# Autodesk Inventor assembly: 000 Ensamblaje hw_LM - BASIC
(part 4 of 4)
- Mate:289: Cooling Kit for NVIDIA Jetson Xavier NX - screws-harness:1 ↔ P3767-pcba-envelop_20230310-modificada:1
## Named parameters: d178_d163 = 0 mm, d193_d188 = 0 mm, d196_d184 = 0 mm, d203_d178_d163 = 0 mm, d205_d180 = 0 mm, d231_d187 = 0 mm, d239_d202_d177_d162 = 0 mm, d304_d302 = 0 mm, d308_d306 = 0 mm, d309_d307 = 0 mm, d310_d304_d302 = 0 mm, d313_d307 = 0 mm, d316_d237_d198_d178_d163 = 0 mm, d317_d238_d200_d180 = 0 mm, d323_d316_d237_d198_d178_d163 = 0 mm, d324_d317_d238_d200_d180 = 0 mm, d325_d318_d240_d203_d178_d163 = 0 mm, d326_d319_d242_d205_d180 = 0 mm, d327_d320_d243_d206 = 0 mm, d328_d321 = 0 mm, d331_d323_d316_d237_d198_d178_d163 = 0 mm, d332_d324_d317_d238_d200_d180 = 0 mm, d337_d322 = 0 mm, d421_d415 = 0 mm, d457_d340 = 0 mm, d464_d457_d340 = 0 mm, d465_d458 = 0 mm, d467_d460 = 0 mm, d471_d456_d340 = 0 mm, d472_d457_d340 = 0 mm, d474_d459 = 0 mm, d477_d463_d456_d340 = 0 mm, d488_d471_d456_d340 = 0 mm, d489_d472_d457_d340 = 0 mm, d490_d473_d458 = 0 mm, d491_d474_d459 = 0 mm, d492_d475_d460 = 0 mm, d493_d476_d461 = 0 mm, d494_d477_d463_d456_d340 = 0 mm, d495_d478_d464_d457_d340 = 0 mm, d496_d479_d465_d458 = 0 mm, d497_d480_d466_d459 = 0 mm, d498_d481_d467_d460 = 0 mm, d499_d482_d468_d461 = 0 mm, d500_d483_d469 = 0 mm, d501_d484_d470 = 0 mm, d502_d486 = 0 mm, d506_d471_d456_d340 = 0 mm, d507_d489_d472_d457_d340 = 0 mm, d508_d490_d473_d458 = 0 mm, d509_d492_d475_d460 = 0 mm, d510_d495_d478_d464_d457_d340 = 0 mm, d511_d496_d479_d465_d458 = 0 mm, d512_d498_d481_d467_d460 = 0 mm, d513_d502_d486 = 0 mm, d514_d503 = 0 mm, d515_d504 = 0 mm, d516_d471_d456_d340 = 0 mm, d520_d495_d478_d464_d457_d340 = 0 mm, d521_d496_d479_d465_d458 = 0 mm, d522_d498_d481_d467_d460 = 0 mm, d524_d503 = 0 mm, d525_d504 = 0 mm, d576_d508_d490_d473_d458 = 0 mm, d591_d581_d575_d507_d489_d472_d457_d340 = 0 mm, d592_d582_d576_d508_d490_d473_d458 = 0 mm, d593_d583_d577_d509_d492_d475_d460 = 0 mm, d594_d584_d578 = 0 mm, d595_d585_d579 = 0 mm, d596_d586_d580 = 0 mm, d597_d589 = 0 mm, d598_d590 = 0 mm, d599_d581_d575_d507_d489_d472_d457_d340 = 0 mm, d600_d582_d576_d508_d490_d473_d458 = 0 mm, d601_d583_d577_d509_d492_d475_d460 = 0 mm, d602_d584_d578 = 0 mm, d603_d585_d579 = 0 mm, d604_d586_d580 = 0 mm, d605_d589 = 0 mm, d606_d590 = 0 mm, d608_d592_d582_d576_d508_d490_d473_d458 = 0 mm, d609_d593_d583_d577_d509_d492_d475_d460 = 0 mm, d611_d595_d585_d579 = 0 mm, d612_d596_d586_d580 = 0 mm, d613_d597_d589 = 0 mm, d614_d598_d590 = 0 mm, d632_d599_d581_d575_d507_d489_d472_d457_d340 = 0 mm, d635_d602_d584_d578 = 0 mm, d638_d605_d589 = 0 mm, d639_d606_d590 = 0 mm, d640_d623 = 0 deg, d644_d627 = 0 deg, d645_d628 = 0 deg, d650_d581_d575_d507_d489_d472_d457_d340 = 0 mm, d651_d582_d576_d508_d490_d473_d458 = 0 mm, d652_d446_d178_d163 = 0 mm, d653_d447_d180 = 0 mm, d654_d449 = 0 mm, d655_d452 = 0 mm, d682_d678 = 0 mm, d683_d679 = 0 mm, d684_d680 = 0 mm, d737_d728 = 0 mm, d738_d730 = 0 mm, d739_d731 = 0 mm, d740_d732 = 0 mm, d746_d737_d728 = 0 mm, d747_d738_d730 = 0 mm, d748_d739_d731 = 0 mm, d749_d740_d732 = 0 mm, d750_d737_d728 = 0 mm, d751_d738_d730 = 0 mm, d752_d739_d731 = 0 mm, d753_d740_d732 = 0 mm, d762_d753_d740_d732 = 0 mm, d766_d753_d740_d732 = 0 mm, d775_d763_d750_d737_d728 = 0 mm, d776_d764_d751_d738_d730 = 0 mm, d777_d765_d752_d739_d731 = 0 mm, d778_d766_d753_d740_d732 = 0 mm, d783_d775_d763_d750_d737_d728 = 0 mm, d784_d777_d765_d752_d739_d731 = 0 mm, d785_d778_d766_d753_d740_d732 = 0 mm, d786_d775_d763_d750_d737_d728 = 0 mm, d787_d777_d765_d752_d739_d731 = 0 mm, d788_d778_d766_d753_d740_d732 = 0 mm, d798_d775_d763_d750_d737_d728 = 0 mm, d799_d786_d775_d763_d750_d737_d728 = 0 mm, d800_d787_d777_d765_d752_d739_d731 = 0 mm, d801_d788_d778_d766_d753_d740_d732 = 0 mm, d802_d790 = 0 deg, d803_d793 = 0 deg, d804_d794 = 0 deg, d810_d786_d775_d763_d750_d737_d728 = 0 mm, d811_d787_d777_d765_d752_d739_d731 = 0 mm, d812_d788_d778_d766_d753_d740_d732 = 0 mm, d814_d793 = 0 deg, d815_d794 = 0 deg, d816_d798_d775_d763_d750_d737_d728 = 0 mm, d817_d799_d786_d775_d763_d750_d737_d728 = 0 mm, d818_d800_d787_d777_d765_d752_d739_d731 = 0 mm, d819_d801_d788_d778_d766_d753_d740_d732 = 0 mm, d820_d802_d790 = 0 deg, d821_d803_d793 = 0 deg, d822_d804_d794 = 0 deg, d823_d805 = 0 mm, d824_d806 = 0 mm, d825_d807 = 0 mm, d836_d829 = 0 mm, d839_d810_d786_d775_d763_d750_d737_d728 = 0 mm, d840_d811_d787_d777_d765_d752_d739_d731 = 0 mm, d841_d812_d788_d778_d766_d753_d740_d732 = 0 mm, d842_d814_d793 = 0 deg, d843_d815_d794 = 0 deg, d844_d817_d799_d786_d775_d763_d750_d737_d728 = 0 mm, d845_d818_d800_d787_d777_d765_d752_d739_d731 = 0 mm, d846_d819_d801_d788_d778_d766_d753_d740_d732 = 0 mm, d847_d821_d803_d793 = 0 deg, d848_d822_d804_d794 = 0 deg, d856_d836_d829 = 0 mm, d857_d837_d775_d763_d750_d737_d728 = 0 mm, d858_d838_d790 = 0 deg, d859_d839_d810_d786_d775_d763_d750_d737_d728 = 0 mm, d860_d840_d811_d787_d777_d765_d752_d739_d731 = 0 mm, d861_d841_d812_d788_d778_d766_d753_d740_d732 = 0 mm, d862_d842_d814_d793 = 0 deg, d863_d843_d815_d794 = 0 deg, d867_d847_d821_d803_d793 = 0 deg, d868_d848_d822_d804_d794 = 0 deg, d870_d851 = 0 mm, d871_d852 = 0 mm, d872_d853 = 0 mm, d886_d883 = 0 mm, d888_d885 = 0 mm, d889_d878 = 0 deg, d890_d880_d878 = 0 deg, d892_d882_d847_d821_d803_d793 = 0 deg, d899_d878 = 0 deg, d901_d847_d821_d803_d793 = 0 deg, d906_d878 = 0 deg, d908_d847_d821_d803_d793 = 0 deg, d1127_d395 = 0 mm, d1128_d396 = 0 mm, d1129_d397 = 0 mm, d1215_d178_d163 = 0 mm, d1216_d180 = 0 mm, d1234_d1229 = 0 mm, d1235_d1230 = 0 mm, d1236_d1231 = 0 mm, d1237_d1232 = 0 mm, d1238_d1233 = 0 mm, d1243_d1241 = 0 mm, d1244_d1242 = 0 mm, d1245_d1229 = 0 mm, d1246_d1230 = 0 mm, d1247_d1231 = 0 mm, d1248_d1232 = 0 mm, d1249_d1233 = 0 mm, d1250_d1234_d1229 = 0 mm, d1251_d1235_d1230 = 0 mm, d1252_d1236_d1231 = 0 mm, d1253_d1237_d1232 = 0 mm, d1254_d1238_d1233 = 0 mm, d1255_d1239 = 0 mm, d1260_d1241 = 0 mm, d1261_d1242 = 0 mm, d1262_d1229 = 0 mm, d1263_d1230 = 0 mm, d1264_d1231 = 0 mm, d1265_d1232 = 0 mm, d1266_d1233 = 0 mm, d1267_d1234_d1229 = 0 mm, d1268_d1235_d1230 = 0 mm, d1269_d1236_d1231 = 0 mm, d1270_d1237_d1232 = 0 mm, d1271_d1238_d1233 = 0 mm, d1272_d1239 = 0 mm, d1273_d1260_d1241 = 0 mm, d1274_d1261_d1242 = 0 mm, d1275_d1262_d1229 = 0 mm, d1276_d1263_d1230 = 0 mm, d1277_d1264_d1231 = 0 mm, d1278_d1265_d1232 = 0 mm, d1279_d1266_d1233 = 0 mm, d1280_d1267_d1234_d1229 = 0 mm, d1281_d1268_d1235_d1230 = 0 mm, d1282_d1269_d1236_d1231 = 0 mm, d1283_d1272_d1239 = 0 mm, d1288_d1260_d1241 = 0 mm, d1289_d1261_d1242 = 0 mm, d1290_d1262_d1229 = 0 mm, d1291_d1263_d1230 = 0 mm, d1292_d1264_d1231 = 0 mm, d1293_d1265_d1232 = 0 mm, d1294_d1266_d1233 = 0 mm, d1295_d1267_d1234_d1229 = 0 mm, d1296_d1268_d1235_d1230 = 0 mm, d1297_d1269_d1236_d1231 = 0 mm, d1298_d1272_d1239 = 0 mm, d1299_d1274_d1261_d1242 = 0 mm, d1300_d1275_d1262_d1229 = 0 mm, d1301_d1276_d1263_d1230 = 0 mm, d1302_d1277_d1264_d1231 = 0 mm, d1303_d1278_d1265_d1232 = 0 mm, d1304_d1279_d1266_d1233 = 0 mm, d1305_d1280_d1267_d1234_d1229 = 0 mm, d1306_d1283_d1272_d1239 = 0 mm, d1307_d1288_d1260_d1241 = 0 mm, d1308_d1289_d1261_d1242 = 0 mm, d1309_d1290_d1262_d1229 = 0 mm, d1310_d1291_d1263_d1230 = 0 mm, d1311_d1292_d1264_d1231 = 0 mm, d1312_d1293_d1265_d1232 = 0 mm, d1313_d1294_d1266_d1233 = 0 mm, d1314_d1295_d1267_d1234_d1229 = 0 mm, d1315_d1296_d1268_d1235_d1230 = 0 mm, d1316_d1297_d1269_d1236_d1231 = 0 mm, d1317_d1298_d1272_d1239 = 0 mm, d1324_d1321 = 0 mm, d1325_d1323 = 0 mm, d1326_d1300_d1275_d1262_d1229 = 0 mm, d1327_d1301_d1276_d1263_d1230 = 0 mm, d1328_d1302_d1277_d1264_d1231 = 0 mm, d1329_d1303_d1278_d1265_d1232 = 0 mm, d1330_d1304_d1279_d1266_d1233 = 0 mm, d1331_d1307_d1288_d1260_d1241 = 0 mm, d1332_d1308_d1289_d1261_d1242 = 0 mm, d1333_d1309_d1290_d1262_d1229 = 0 mm, d1334_d1310_d1291_d1263_d1230 = 0 mm, d1335_d1311_d1292_d1264_d1231 = 0 mm, d1336_d1312_d1293_d1265_d1232 = 0 mm, d1337_d1313_d1294_d1266_d1233 = 0 mm, d1338_d1314_d1295_d1267_d1234_d1229 = 0 mm, d1339_d1315_d1296_d1268_d1235_d1230 = 0 mm, d1340_d1316_d1297_d1269_d1236_d1231 = 0 mm, d1341_d1317_d1298_d1272_d1239 = 0 mm, d1350_d1324_d1321 = 0 mm, d1351_d1325_d1323 = 0 mm, d1352_d1326_d1300_d1275_d1262_d1229 = 0 mm, d1353_d1327_d1301_d1276_d1263_d1230 = 0 mm, d1354_d1328_d1302_d1277_d1264_d1231 = 0 mm, d1355_d1329_d1303_d1278_d1265_d1232 = 0 mm, d1356_d1330_d1304_d1279_d1266_d1233 = 0 mm, d1357_d1331_d1307_d1288_d1260_d1241 = 0 mm, d1358_d1332_d1308_d1289_d1261_d1242 = 0 mm, d1359_d1333_d1309_d1290_d1262_d1229 = 0 mm, d1360_d1334_d1310_d1291_d1263_d1230 = 0 mm, d1361_d1335_d1311_d1292_d1264_d1231 = 0 mm, d1362_d1336_d1312_d1293_d1265_d1232 = 0 mm, d1363_d1337_d1313_d1294_d1266_d1233 = 0 mm, d1364_d1338_d1314_d1295_d1267_d1234_d1229 = 0 mm, d1365_d1339_d1315_d1296_d1268_d1235_d1230 = 0 mm, d1366_d1340_d1316_d1297_d1269_d1236_d1231 = 0 mm, d1367_d1341_d1317_d1298_d1272_d1239 = 0 mm, d1370_d1363_d1337_d1313_d1294_d1266_d1233 = 0 mm, d1377_d1370_d1363_d1337_d1313_d1294_d1266_d1233 = 0 mm, d1378_d1372 = 0 deg, d1379_d1373 = 0 deg, d1380_d1374 = 0 mm, d1381_d1375 = 0 mm, d1382_d1370_d1363_d1337_d1313_d1294_d1266_d1233 = 0 mm, d1383_d1372 = 0 deg, d1384_d1373 = 0 deg, d1385_d1374 = 0 mm, d1386_d1375 = 0 mm, d1391_d1370_d1363_d1337_d1313_d1294_d1266_d1233 = 0 mm, d1392_d1372 = 0 deg, d1393_d1373 = 0 deg, d1394_d1374 = 0 mm, d1395_d1375 = 0 mm, d1397_d1378_d1372 = 0 deg, d1398_d1379_d1373 = 0 deg, d1399_d1380_d1374 = 0 mm, d1400_d1381_d1375 = 0 mm, d1402_d1383_d1372 = 0 deg, d1403_d1384_d1373 = 0 deg, d1404_d1385_d1374 = 0 mm, d1405_d1386_d1375 = 0 mm, d1406_d1387 = 0 mm, d1407_d1388 = 0 mm, d1408_d1389 = 0 mm, d1409_d1390 = 0 mm, d1410_d1370_d1363_d1337_d1313_d1294_d1266_d1233 = 0 mm, d1411_d1372 = 0 deg, d1412_d1373 = 0 deg, d1413_d1374 = 0 mm, d1414_d1375 = 0 mm, d1416_d1378_d1372 = 0 deg, d1417_d1379_d1373 = 0 deg, d1418_d1380_d1374 = 0 mm, d1419_d1381_d1375 = 0 mm, d1421_d1383_d1372 = 0 deg, d1422_d1384_d1373 = 0 deg, d1423_d1385_d1374 = 0 mm, d1424_d1386_d1375 = 0 mm, d1425_d1387 = 0 mm, d1426_d1388 = 0 mm, d1427_d1389 = 0 mm, d1428_d1390 = 0 mm, d1433_d1411_d1372 = 0 deg, d1434_d1412_d1373 = 0 deg, d1435_d1413_d1374 = 0 mm, d1436_d1414_d1375 = 0 mm, d1438_d1416_d1378_d1372 = 0 deg, d1439_d1417_d1379_d1373 = 0 deg, d1440_d1418_d1380_d1374 = 0 mm, d1441_d1419_d1381_d1375 = 0 mm, d1443_d1421_d1383_d1372 = 0 deg, d1444_d1422_d1384_d1373 = 0 deg, d1445_d1423_d1385_d1374 = 0 mm, d1446_d1424_d1386_d1375 = 0 mm, d1447_d1425_d1387 = 0 mm, d1448_d1426_d1388 = 0 mm, d1449_d1427_d1389 = 0 mm, d1450_d1428_d1390 = 0 mm, d1452_d1411_d1372 = 0 deg, d1453_d1412_d1373 = 0 deg, d1454_d1413_d1374 = 0 mm, d1455_d1414_d1375 = 0 mm, d1457_d1416_d1378_d1372 = 0 deg, d1458_d1417_d1379_d1373 = 0 deg, d1459_d1418_d1380_d1374 = 0 mm, d1460_d1419_d1381_d1375 = 0 mm, d1462_d1421_d1383_d1372 = 0 deg, d1463_d1422_d1384_d1373 = 0 deg, d1464_d1423_d1385_d1374 = 0 mm, d1465_d1424_d1386_d1375 = 0 mm, d1466_d1425_d1387 = 0 mm, d1467_d1426_d1388 = 0 mm, d1468_d1427_d1389 = 0 mm, d1469_d1428_d1390 = 0 mm, d1474_d1433_d1411_d1372 = 0 deg, d1475_d1434_d1412_d1373 = 0 deg, d1476_d1435_d1413_d1374 = 0 mm, d1477_d1436_d1414_d1375 = 0 mm, d1479_d1438_d1416_d1378_d1372 = 0 deg, d1480_d1439_d1417_d1379_d1373 = 0 deg, d1481_d1440_d1418_d1380_d1374 = 0 mm, d1482_d1441_d1419_d1381_d1375 = 0 mm, d1484_d1443_d1421_d1383_d1372 = 0 deg, d1485_d1444_d1422_d1384_d1373 = 0 deg, d1486_d1445_d1423_d1385_d1374 = 0 mm, d1487_d1446_d1424_d1386_d1375 = 0 mm, d1488_d1447_d1425_d1387 = 0 mm, d1489_d1448_d1426_d1388 = 0 mm, d1490_d1449_d1427_d1389 = 0 mm, d1491_d1450_d1428_d1390 = 0 mm, d1493_d1433_d1411_d1372 = 0 deg, d1494_d1434_d1412_d1373 = 0 deg, d1495_d1435_d1413_d1374 = 0 mm, d1496_d1436_d1414_d1375 = 0 mm, d1498_d1438_d1416_d1378_d1372 = 0 deg, d1499_d1439_d1417_d1379_d1373 = 0 deg, d1500_d1440_d1418_d1380_d1374 = 0 mm, d1501_d1441_d1419_d1381_d1375 = 0 mm, d1503_d1443_d1421_d1383_d1372 = 0 deg, d1504_d1444_d1422_d1384_d1373 = 0 deg, d1505_d1445_d1423_d1385_d1374 = 0 mm, d1506_d1446_d1424_d1386_d1375 = 0 mm, d1507_d1447_d1425_d1387 = 0 mm, d1508_d1448_d1426_d1388 = 0 mm, d1509_d1449_d1427_d1389 = 0 mm, d1510_d1450_d1428_d1390 = 0 mm, d1516_d1493_d1433_d1411_d1372 = 0 deg, d1517_d1494_d1434_d1412_d1373 = 0 deg, d1518_d1495_d1435_d1413_d1374 = 0 mm, d1519_d1496_d1436_d1414_d1375 = 0 mm, d1521_d1498_d1438_d1416_d1378_d1372 = 0 deg, d1522_d1499_d1439_d1417_d1379_d1373 = 0 deg, d1523_d1500_d1440_d1418_d1380_d1374 = 0 mm, d1524_d1501_d1441_d1419_d1381_d1375 = 0 mm, d1526_d1503_d1443_d1421_d1383_d1372 = 0 deg, d1527_d1504_d1444_d1422_d1384_d1373 = 0 deg, d1528_d1505_d1445_d1423_d1385_d1374 = 0 mm, d1529_d1506_d1446_d1424_d1386_d1375 = 0 mm, d1530_d1507_d1447_d1425_d1387 = 0 mm, d1531_d1508_d1448_d1426_d1388 = 0 mm, d1532_d1509_d1449_d1427_d1389 = 0 mm, d1533_d1510_d1450_d1428_d1390 = 0 mm, d1535_d1493_d1433_d1411_d1372 = 0 deg, d1536_d1494_d1434_d1412_d1373 = 0 deg, d1537_d1495_d1435_d1413_d1374 = 0 mm, d1538_d1496_d1436_d1414_d1375 = 0 mm, d1540_d1498_d1438_d1416_d1378_d1372 = 0 deg, d1541_d1499_d1439_d1417_d1379_d1373 = 0 deg, d1542_d1500_d1440_d1418_d1380_d1374 = 0 mm, d1543_d1501_d1441_d1419_d1381_d1375 = 0 mm, d1545_d1503_d1443_d1421_d1383_d1372 = 0 deg, d1546_d1504_d1444_d1422_d1384_d1373 = 0 deg, d1547_d1505_d1445_d1423_d1385_d1374 = 0 mm, d1548_d1506_d1446_d1424_d1386_d1375 = 0 mm, d1549_d1507_d1447_d1425_d1387 = 0 mm, d1550_d1508_d1448_d1426_d1388 = 0 mm, d1551_d1509_d1449_d1427_d1389 = 0 mm, d1552_d1510_d1450_d1428_d1390 = 0 mm, d1559_d1521_d1498_d1438_d1416_d1378_d1372 = 0 deg, d1561_d1526_d1503_d1443_d1421_d1383_d1372 = 0 deg, d1562_d1527_d1504_d1444_d1422_d1384_d1373 = 0 deg, d1563_d1528_d1505_d1445_d1423_d1385_d1374 = 0 mm, d1564_d1529_d1506_d1446_d1424_d1386_d1375 = 0 mm, d1565_d1533_d1510_d1450_d1428_d1390 = 0 mm, d1567_d1493_d1433_d1411_d1372 = 0 deg, d1568_d1494_d1434_d1412_d1373 = 0 deg, d1569_d1495_d1435_d1413_d1374 = 0 mm, d1570_d1496_d1436_d1414_d1375 = 0 mm, d1572_d1498_d1438_d1416_d1378_d1372 = 0 deg, d1573_d1499_d1439_d1417_d1379_d1373 = 0 deg, d1574_d1500_d1440_d1418_d1380_d1374 = 0 mm, d1575_d1501_d1441_d1419_d1381_d1375 = 0 mm, d1577_d1503_d1443_d1421_d1383_d1372 = 0 deg, d1578_d1504_d1444_d1422_d1384_d1373 = 0 deg, d1579_d1505_d1445_d1423_d1385_d1374 = 0 mm, d1580_d1506_d1446_d1424_d1386_d1375 = 0 mm, d1581_d1507_d1447_d1425_d1387 = 0 mm, d1582_d1508_d1448_d1426_d1388 = 0 mm, d1583_d1509_d1449_d1427_d1389 = 0 mm, d1584_d1510_d1450_d1428_d1390 = 0 mm, d1585_d1557 = 0 mm, d1586_d1558 = 0 mm, d1591_d1521_d1498_d1438_d1416_d1378_d1372 = 0 deg, d1593_d1526_d1503_d1443_d1421_d1383_d1372 = 0 deg, d1594_d1527_d1504_d1444_d1422_d1384_d1373 = 0 deg, d1595_d1528_d1505_d1445_d1423_d1385_d1374 = 0 mm, d1596_d1529_d1506_d1446_d1424_d1386_d1375 = 0 mm, d1597_d1533_d1510_d1450_d1428_d1390 = 0 mm, d1598_d1582_d1508_d1448_d1426_d1388 = 0 mm, d1599_d1583_d1509_d1449_d1427_d1389 = 0 mm, d1600_d1584_d1510_d1450_d1428_d1390 = 0 mm, d1601_d1588 = 0 mm, d1602_d1590 = 0 mm, d1604_d1567_d1493_d1433_d1411_d1372 = 0 deg, d1605_d1568_d1494_d1434_d1412_d1373 = 0 deg, d1606_d1569_d1495_d1435_d1413_d1374 = 0 mm, d1607_d1570_d1496_d1436_d1414_d1375 = 0 mm, d1609_d1572_d1498_d1438_d1416_d1378_d1372 = 0 deg, d1610_d1573_d1499_d1439_d1417_d1379_d1373 = 0 deg, d1611_d1574_d1500_d1440_d1418_d1380_d1374 = 0 mm, d1612_d1575_d1501_d1441_d1419_d1381_d1375 = 0 mm, d1614_d1577_d1503_d1443_d1421_d1383_d1372 = 0 deg, d1615_d1578_d1504_d1444_d1422_d1384_d1373 = 0 deg, d1616_d1579_d1505_d1445_d1423_d1385_d1374 = 0 mm, d1617_d1580_d1506_d1446_d1424_d1386_d1375 = 0 mm, d1618_d1581_d1507_d1447_d1425_d1387 = 0 mm, d1622_d1598_d1582_d1508_d1448_d1426_d1388 = 0 mm, d1623_d1600_d1584_d1510_d1450_d1428_d1390 = 0 mm, d1624_d1604_d1567_d1493_d1433_d1411_d1372 = 0 deg, d1626_d1609_d1572_d1498_d1438_d1416_d1378_d1372 = 0 deg, d1627_d1610_d1573_d1499_d1439_d1417_d1379_d1373 = 0 deg, d1628_d1611_d1574_d1500_d1440_d1418_d1380_d1374 = 0 mm, d1629_d1612_d1575_d1501_d1441_d1419_d1381_d1375 = 0 mm, d1631_d1614_d1577_d1503_d1443_d1421_d1383_d1372 = 0 deg, d1632_d1615_d1578_d1504_d1444_d1422_d1384_d1373 = 0 deg, d1633_d1616_d1579_d1505_d1445_d1423_d1385_d1374 = 0 mm, d1634_d1617_d1580_d1506_d1446_d1424_d1386_d1375 = 0 mm, d1635_d1618_d1581_d1507_d1447_d1425_d1387 = 0 mm, d1638_d1622_d1598_d1582_d1508_d1448_d1426_d1388 = 0 mm, d1639_d1623_d1600_d1584_d1510_d1450_d1428_d1390 = 0 mm, d1640_d1624_d1604_d1567_d1493_d1433_d1411_d1372 = 0 deg, d1651_d1635_d1618_d1581_d1507_d1447_d1425_d1387 = 0 mm, d1652_d1622_d1598_d1582_d1508_d1448_d1426_d1388 = 0 mm, d1653_d1623_d1600_d1584_d1510_d1450_d1428_d1390 = 0 mm, d1654_d1624_d1604_d1567_d1493_d1433_d1411_d1372 = 0 deg, d1665_d1635_d1618_d1581_d1507_d1447_d1425_d1387 = 0 mm, d1729_d1727 = 0 mm, d1737_d1734 = 0 mm, d1738_d1736 = 0 mm, d1739_d1734 = 0 mm, d1740_d1736 = 0 mm, d1741_d1734 = 0 mm, d1742_d1736 = 0 mm, d1747_d1743 = 0 mm, d1748_d1737_d1734 = 0 mm, d1749_d1738_d1736 = 0 mm, d1750_d1739_d1734 = 0 mm, d1751_d1740_d1736 = 0 mm, d1758_d1754 = 0 mm, d1760_d1758_d1754 = 0 mm, d1770_d1766 = 0 mm, d1776_d1775 = 0 mm, d1777_d1774 = 0 mm, d1778_d1775 = 0 mm, d1779_d1774 = 0 mm, d1787_d746_d737_d728 = 0 mm, d1802_d1775 = 0 mm, d1803_d1774 = 0 mm
